# Autodesk Inventor assembly: ModuleBase
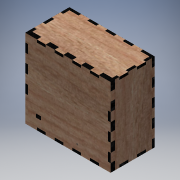
[picture p0: Inventor's stored thumbnail of the model, 180x180]
Saved by Autodesk Inventor 2019.4 (Build 234330000, 330)
## iProperties
Created: 2020-06-30
Part Number: ModuleBase
Document SubType Name: Assembly
Designer: wimva
Author: wimva
## Documents named in this file (6)
- C:\Users\wimva\source\repos\BombSquad\Mechanical\Modules\ModuleBase.iam
- C:\Users\wimva\source\repos\BombSquad\Mechanical\Modules\FrontPlateBase.ipt
- C:\Users\wimva\source\repos\BombSquad\Mechanical\Modules\BackPlateBase.ipt
- C:\Users\wimva\source\repos\BombSquad\Mechanical\Modules\LeftRightPlate.ipt
- C:\Users\wimva\source\repos\BombSquad\Mechanical\Modules\TopBottomPlate.ipt
- C:\Users\wimva\source\repos\BombSquad\Mechanical\Modules\Dimensions.xlsx
## Components (6 placed, 5 different names)
1. FrontPlate — Mate:4, Flush:1, Flush:2, Mate:5, Flush:6, Flush:7, Flush:8, Flush:10, Mate:6, Mate:7, Flush:13
2. BackPlate — Mate:1, Mate:2, Mate:3, Mate:4, Flush:1, Flush:2, Flush:9, Flush:15
3. LeftPlate — Mate:5, Flush:9, Flush:10, Flush:14, Flush:16
4. RightPlate — Flush:6, Flush:7, Flush:8
5. TopBottomPlate:1 — Mate:7, Flush:13, Flush:14
6. TopBottomPlate:2 — Mate:6, Flush:15, Flush:16
## Relationships (18: Flush 11, Mate 7)
- Mate:1: BackPlate
- Mate:2: BackPlate
- Mate:3: BackPlate
- Mate:4 (-50 mm): FrontPlate ↔ BackPlate
- Flush:1: FrontPlate ↔ BackPlate
- Flush:2: FrontPlate ↔ BackPlate
- Mate:5: FrontPlate ↔ LeftPlate
- Flush:6: FrontPlate ↔ RightPlate
- Flush:7: FrontPlate ↔ RightPlate
- Flush:8: FrontPlate ↔ RightPlate
- Flush:9: BackPlate ↔ LeftPlate
- Flush:10: FrontPlate ↔ LeftPlate
- Mate:6: FrontPlate ↔ TopBottomPlate:2
- Mate:7: FrontPlate ↔ TopBottomPlate:1
- Flush:13: FrontPlate ↔ TopBottomPlate:1
- Flush:14: LeftPlate ↔ TopBottomPlate:1
- Flush:15: BackPlate ↔ TopBottomPlate:2
- Flush:16: LeftPlate ↔ TopBottomPlate:2
## Named parameters: RackWidth = 482.6 mm, U = 44.5 mm, Module_Width = 96.52 mm, Module_Height = 89 mm, Module_Depth = 50 mm, Module_Case_Thickness = 3 mm, Module_Back_Thickness = 5 mm, Module_Case_SlotDepth = 3 mm, Module_Case_SlotWidth = 10 mm, Module_Connector_Width = 6 mm, Module_Connector_Depth = 4 mm, Module_StatusIndicatorDiameter = 5 mm, Module_Case_BottomSlotDepth = 5 mm
